# Autodesk Inventor assembly: m4 bearing assembly 30mm
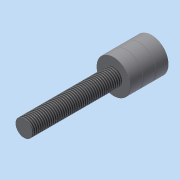
[picture p0: Inventor's stored thumbnail of the model, 180x180]
Saved by Autodesk Inventor 2015 (Build 190159000, 159)
## iProperties
Created: 2016-09-08
Part Number: m4 bearing assembly 30mm
Document SubType Name: Assembly
Designer: Dustin
Author: Dustin
## Documents named in this file (3)
- E:\Documents\3D Printer\Parts\New Printer\m4 bearing assembly 30mm.iam
- E:\Documents\3D Printer\Parts\New Printer\8x4x3 bearing.ipt
- E:\Documents\3D Printer\Parts\New Printer\m4x30.ipt
## Components (4 placed, 2 different names)
1. 8x4x3 bearing:1 — Mate:3, Insert:3
2. 8x4x3 bearing:2 — Mate:2, Mate:3, Insert:2, Insert:3
3. 8x4x3 bearing:3 — Mate:2, Insert:1, Insert:2
4. m4x30:1 — Insert:1
## Relationships (5: Insert 3, Mate 2)
- Mate:2: 8x4x3 bearing:2 ↔ 8x4x3 bearing:3
- Mate:3: 8x4x3 bearing:1 ↔ 8x4x3 bearing:2
- Insert:1: 8x4x3 bearing:3 ↔ m4x30:1
- Insert:2: 8x4x3 bearing:2 ↔ 8x4x3 bearing:3
- Insert:3: 8x4x3 bearing:1 ↔ 8x4x3 bearing:2
